# Autodesk Inventor assembly: Robot!
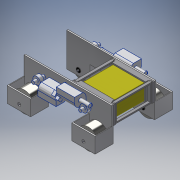
[picture p0: Inventor's stored thumbnail of the model, 180x180]
Saved by Autodesk Inventor 2016 (Build 200138000, 138)
## iProperties
Created: 2015-11-03
Part Number: Robot!
Document SubType Name: Assembly
Designer: rossmosier
Author: rossmosier
## Documents named in this file (7)
- C:\Users\rossmosier\Documents\CAD Team\CADTeam\Assemblies\Robot!.iam
- C:\Users\rossmosier\Documents\CAD Team\CADTeam\Parts\Brain.ipt
- C:\Users\rossmosier\Documents\CAD Team\CADTeam\Drive Train\driveAssembly.iam
- C:\Users\rossmosier\Documents\CAD Team\CADTeam\Parts\doveTailSide.ipt
- C:\Users\rossmosier\Documents\CAD Team\CADTeam\Parts\doveTailOtherSide.ipt
- C:\Users\rossmosier\Documents\CAD Team\CADTeam\Drive Train\driveAssembly_MIR1.iam
- C:\Users\rossmosier\Documents\CAD Team\CADTeam\Parts\doveTailBar.ipt
## Components (7 placed, 6 different names)
1. driveAssembly:1 [sub-assembly] — Mate:1, Mate:2
2. doveTailOtherSide:1 — Mate:1, Mate:8, Mate:9
3. Brain:1 — Mate:2, Mate:3, Mate:4, Mate:5, Mate:6
4. doveTailSide:1 — Mate:3, Mate:7
5. driveAssembly_MIR1:1 [sub-assembly] — Mate:7
6. doveTailBar:1 — Mate:8
7. doveTailBar:2 — Mate:9
## Relationships (9: Mate 9)
- Mate:1: driveAssembly:1 ↔ doveTailOtherSide:1
- Mate:2: driveAssembly:1 ↔ Brain:1
- Mate:3: Brain:1 ↔ doveTailSide:1
- Mate:4: Brain:1
- Mate:5: Brain:1
- Mate:6: Brain:1
- Mate:7: doveTailSide:1 ↔ driveAssembly_MIR1:1
- Mate:8: doveTailOtherSide:1 ↔ doveTailBar:1
- Mate:9: doveTailOtherSide:1 ↔ doveTailBar:2
